# Autodesk Inventor assembly: Hikvision_DS-U02
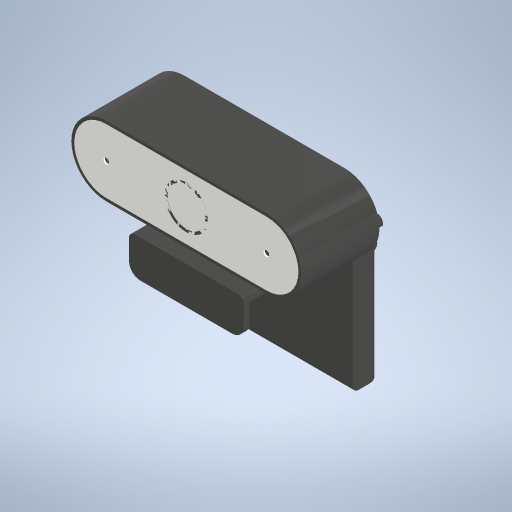
[picture p0: Inventor's stored thumbnail of the model, 512x512]
Saved by Autodesk Inventor 2024 (Build 280153000, 153)
## iProperties
Created: 2022-01-03
Part Number: Hikvision_DS-U02
Document SubType Name: Assembly
Designer: ASUS
Sending System: Autodesk Translation Framework v10.10.0.1391
Preprocessor: ST-DEVELOPER v18.1
Title: C:/Users/lippi/3D Objects/Hikvision_DS-U02.step
## Documents named in this file (4)
- C:\Users\ASUS\OneDrive\Dokumen\TUGAS\WebCam\Hikvision_DS-U02.iam
- C:\Users\ASUS\OneDrive\Dokumen\TUGAS\WebCam\camera.ipt
- C:\Users\ASUS\OneDrive\Dokumen\TUGAS\WebCam\holder.ipt
- C:\Users\ASUS\OneDrive\Dokumen\TUGAS\WebCam\down_holder.ipt
## Components (3 placed, 3 different names)
1. camera:1
2. holder:1 — Mate:1, Flush:1
3. down_holder:1 — Mate:1, Flush:1
## Relationships (2: Mate 1, Flush 1)
- Mate:1: holder:1 ↔ down_holder:1
- Flush:1: holder:1 ↔ down_holder:1
